# Autodesk Inventor assembly: Montagem2
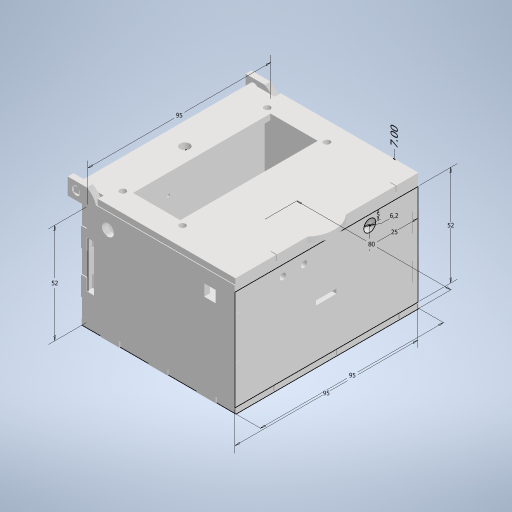
[picture p0: Inventor's stored thumbnail of the model, 512x512]
Saved by Autodesk Inventor 2024 (Build 280153000, 153)
## iProperties
Created: 2023-12-01
Part Number: Montagem2
Document SubType Name: Assembly
Designer: caiot
Author: caiot
## Documents named in this file (7)
- C:\Users\caiot\OneDrive\Documentos\IPT_CASE\Montagem2.iam
- C:\Users\caiot\OneDrive\Documentos\IPT_CASE\Fundo.ipt
- C:\Users\caiot\OneDrive\Documentos\IPT_CASE\Parede_HX711.ipt
- C:\Users\caiot\OneDrive\Documentos\IPT_CASE\Tampa.ipt
- C:\Users\caiot\OneDrive\Documentos\IPT_CASE\Parede_lateral_3.ipt
- C:\Users\caiot\OneDrive\Documentos\IPT_CASE\Parede_lateral_2.ipt
- C:\Users\caiot\OneDrive\Documentos\IPT_CASE\Parede_lateral_1.ipt
## Components (6 placed, 6 different names)
1. Fundo:1 — Alinhado:1, Alinhado:2, Coincidente:1, Alinhado:3, Alinhado:4, Coincidente:2, Alinhado:5, Alinhado:7, Coincidente:3, Alinhado:9, Coincidente:4
2. Parede_lateral_3:1 — Alinhado:1, Alinhado:2, Coincidente:1, Alinhado:6
3. Parede_HX711:1 — Alinhado:3, Alinhado:4, Coincidente:2, Alinhado:10
4. Parede_lateral_2:1 — Alinhado:5, Alinhado:6, Alinhado:7, Coincidente:3, Alinhado:8, Coincidente:5
5. Parede_lateral_1:1 — Alinhado:8, Alinhado:9, Coincidente:4, Alinhado:11
6. Tampa:1 — Alinhado:10, Alinhado:11, Coincidente:5
## Relationships (16: Flush 11, Mate 5)
- Alinhado:1 [Flush]: Fundo:1 ↔ Parede_lateral_3:1
- Alinhado:2 [Flush]: Fundo:1 ↔ Parede_lateral_3:1
- Coincidente:1 [Mate]: Fundo:1 ↔ Parede_lateral_3:1
- Alinhado:3 [Flush]: Fundo:1 ↔ Parede_HX711:1
- Alinhado:4 [Flush]: Fundo:1 ↔ Parede_HX711:1
- Coincidente:2 [Mate]: Fundo:1 ↔ Parede_HX711:1
- Alinhado:5 [Flush]: Fundo:1 ↔ Parede_lateral_2:1
- Alinhado:6 [Flush]: Parede_lateral_3:1 ↔ Parede_lateral_2:1
- Alinhado:7 [Flush]: Fundo:1 ↔ Parede_lateral_2:1
- Coincidente:3 [Mate]: Fundo:1 ↔ Parede_lateral_2:1
- Alinhado:8 [Flush]: Parede_lateral_2:1 ↔ Parede_lateral_1:1
- Alinhado:9 [Flush]: Fundo:1 ↔ Parede_lateral_1:1
- Coincidente:4 [Mate]: Fundo:1 ↔ Parede_lateral_1:1
- Alinhado:10 [Flush]: Parede_HX711:1 ↔ Tampa:1
- Alinhado:11 [Flush]: Parede_lateral_1:1 ↔ Tampa:1
- Coincidente:5 [Mate]: Parede_lateral_2:1 ↔ Tampa:1
